# Autodesk Inventor assembly: POM_T5_04
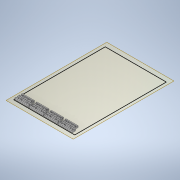
[picture p0: Inventor's stored thumbnail of the model, 180x180]
Saved by Autodesk Inventor 2022.3 (Build 263350000, 350)
## iProperties
Created: 2022-09-28
Part Number: POM_T5_04
Document SubType Name: Assembly
Designer: Masato
Author: Masato
## Documents named in this file (4)
- C:\Users\Masato\Documents\Inventor\Inventor for CIT Brains\SUSTAINA-OP - cam\Cam\POM_T5\OriginalMind_SR420\POM_T5_04.iam
- C:\Users\Masato\Documents\Inventor\Inventor for CIT Brains\SUSTAINA-OP - cam\Cam\DisposableBoard.ipt
- C:\Users\Masato\Documents\Inventor\Inventor for CIT Brains\SUSTAINA-OP - cam\OptionParts\DrillingJigs\Trunk_chest_frame_Jig_side.ipt
- C:\Users\Masato\Documents\Inventor\Inventor for CIT Brains\SUSTAINA-OP - cam\OptionParts\DrillingJigs\Trunk_chest_frame_Jig_top.ipt
## Components (9 placed, 3 different names)
1. DisposableBoard:1 — フラッシュ:1, フラッシュ:2, フラッシュ:3, フラッシュ:4, フラッシュ:5, フラッシュ:6
2. Trunk_chest_frame_Jig_side:1 — メイト:1, フラッシュ:5, フラッシュ:6, フラッシュ:7, メイト:3
3. Trunk_chest_frame_Jig_top:1 — メイト:2, フラッシュ:7, メイト:3
4. Trunk_chest_frame_Jig_side:2
5. Trunk_chest_frame_Jig_top:2
6. Trunk_chest_frame_Jig_side:3
7. Trunk_chest_frame_Jig_top:3
8. Trunk_chest_frame_Jig_side:4
9. Trunk_chest_frame_Jig_top:4
## Component patterns: (4 elements, first: Trunk_chest_frame_Jig_side:1 + Trunk_chest_frame_Jig_top:1)
## Relationships (10: Flush 7, Mate 3)
- フラッシュ:1 [Flush]: DisposableBoard:1
- フラッシュ:2 [Flush]: DisposableBoard:1
- フラッシュ:3 [Flush]: DisposableBoard:1
- フラッシュ:4 [Flush]: DisposableBoard:1
- メイト:1 [Mate]: Trunk_chest_frame_Jig_side:1
- メイト:2 [Mate]: Trunk_chest_frame_Jig_top:1
- フラッシュ:5 [Flush] (2 mm): DisposableBoard:1 ↔ Trunk_chest_frame_Jig_side:1
- フラッシュ:6 [Flush] (-2 mm): DisposableBoard:1 ↔ Trunk_chest_frame_Jig_side:1
- フラッシュ:7 [Flush]: Trunk_chest_frame_Jig_side:1 ↔ Trunk_chest_frame_Jig_top:1
- メイト:3 [Mate] (2.1 mm): Trunk_chest_frame_Jig_side:1 ↔ Trunk_chest_frame_Jig_top:1
